# Autodesk Inventor assembly: Assembly of Polar Express [Copy]
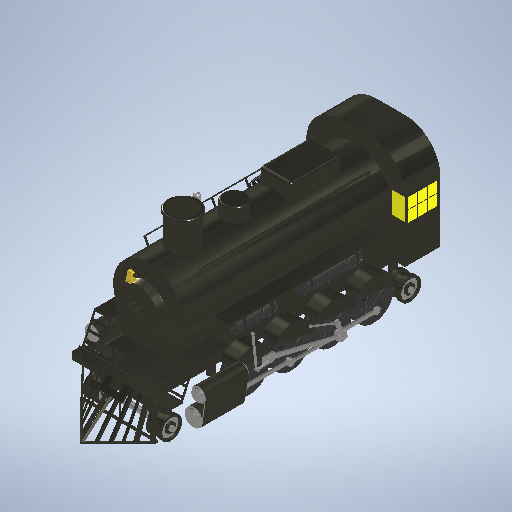
[picture p0: Inventor's stored thumbnail of the model, 512x512]
Saved by Autodesk Inventor 2025.1 (Build 291241020, 241B)
## iProperties
Created: 2022-11-21
Part Number: Assembly of Polar Express [Copy]
Document SubType Name: Assembly
Designer: mc_vlongo24
Author: mc_vlongo24
## Documents named in this file (9)
- C:\Users\Vinny\Downloads\Assembly of Polar Express [Copy].iam
- C:\Users\Vinny\Downloads\Polar Express Start.ipt
- C:\Users\Vinny\Downloads\Stack of train.ipt
- C:\Users\Vinny\Downloads\Cow Catcher of train.ipt
- C:\Users\Vinny\Downloads\Hitch to the Polar Express.ipt
- C:\Users\Vinny\Downloads\Big wheel of Polar Express.ipt
- C:\Users\Vinny\Downloads\Linkage Arms.ipt
- C:\Users\Vinny\Downloads\Small Wheels for Polar Express.ipt
- C:\Users\Vinny\Downloads\Wheel Holder of Train.ipt
## Components (12 placed, 8 different names)
1. Polar Express Start:1 — Insert:1, Mate:1, Insert:2, Flush:1
2. Stack of train:1 — Insert:1
3. Cow Catcher of train:1 — Mate:1
4. Hitch to the Polar Express:1 — Insert:2
5. Big wheel of Polar Express:1 — Mate:3
6. Big wheel of Polar Express:2
7. Big wheel of Polar Express:3
8. Big wheel of Polar Express:4 — Mate:2
9. Linkage Arms:1 — Mate:2, Mate:3
10. Small Wheels for Polar Express:1
11. Small Wheels for Polar Express:2
12. Wheel Holder of Train:1
## Relationships (6: Mate 3, Insert 2, Flush 1)
- Insert:1: Polar Express Start:1 ↔ Stack of train:1
- Mate:1: Polar Express Start:1 ↔ Cow Catcher of train:1
- Insert:2: Polar Express Start:1 ↔ Hitch to the Polar Express:1
- Mate:2: Big wheel of Polar Express:4 ↔ Linkage Arms:1
- Mate:3: Big wheel of Polar Express:1 ↔ Linkage Arms:1
- Flush:1: Polar Express Start:1
